# Autodesk Inventor assembly: Synchronous Belts Transmission
Saved by Autodesk Inventor 2016 (Build 200138000, 138)
## iProperties
Created: 2015-05-19
Part Number: Synchronous Belts Transmission
Document SubType Name: Assembly
Designer: as
Mass: 64.5257 g
Surface Area: 371.595 cm^2
Volume: 21.6802 cm^3
Density: 2.97625 g/cm^3
ClientObjectVersion: 1
Author: as
## Documents named in this file (4)
- C:\Users\as\Documents\Inventor\mintplacer-export\X-portal-assembly-LWLF42\Design Accelerator\Synchronous Belts Transmission2.iam
- C:\Users\as\Documents\Inventor\mintplacer-export\X-portal-assembly-LWLF42\Design Accelerator\Synchronous Belt2.ipt
- C:\Users\as\Documents\Inventor\mintplacer-export\X-portal-assembly-LWLF42\Design Accelerator\Synchronous Pulley12.ipt
- C:\Users\as\Documents\Inventor\mintplacer-export\X-portal-assembly-LWLF42\Design Accelerator\Synchronous Pulley22.ipt
## Components (3 placed, 3 different names)
1. Synchronous Belt:1 — Flush:1, Mate:1, Mate:2, Flush:2, Mate:3, Mate:4
2. Synchronous Pulley1:1 — Flush:1, Mate:1, Mate:2, Rotation:1
3. Synchronous Pulley2:1 — Flush:2, Mate:3, Rotation:1, Mate:4
## Relationships (7: Mate 4, Flush 2, RelateRotation 1)
- Flush:1: Synchronous Belt:1 ↔ Synchronous Pulley1:1
- Mate:1: Synchronous Belt:1 ↔ Synchronous Pulley1:1
- Mate:2: Synchronous Belt:1 ↔ Synchronous Pulley1:1
- Flush:2: Synchronous Belt:1 ↔ Synchronous Pulley2:1
- Mate:3: Synchronous Belt:1 ↔ Synchronous Pulley2:1
- Rotation:1 [RelateRotation] (1 ul): Synchronous Pulley1:1 ↔ Synchronous Pulley2:1
- Mate:4: Synchronous Belt:1 ↔ Synchronous Pulley2:1
